# Autodesk Inventor assembly: Tamale Assembly Plate 0p625in with PCB
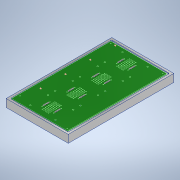
[picture p0: Inventor's stored thumbnail of the model, 180x180]
Saved by Autodesk Inventor 2022 (Build 260153000, 153)
## iProperties
Created: 2022-01-14
Part Number: Tamale Assembly Plate 0p625in with PCB
Document SubType Name: Assembly
Designer: Caleb
Author: Caleb
## Documents named in this file (3)
- C:\Users\Caleb\Desktop\nebraska-silicon-lab\Hardware\ETL\Module Assembly\Tamale Assembly Plate V2\Tamale Assembly Plate 0p625in with PCB.iam
- C:\Users\Caleb\Desktop\nebraska-silicon-lab\Hardware\ETL\Module Assembly\Tamale Assembly Plate V2\Tamale Assembly Plate 0p625in.ipt
- C:\Users\Caleb\Desktop\nebraska-silicon-lab\Hardware\ETL\Module Assembly\Tamale Assembly Plate V2\etl_assembly_plate_pcb_v1.1\etl_assembly_plate_pcb_v1.iam
## Components (2 placed, 2 different names)
1. Tamale Assembly Plate 0p625in:1 — Mate:1, Angle:1, Insert:1
2. etl_assembly_plate_pcb_v1:1 [sub-assembly] — Mate:1, Angle:1, Insert:1
## Relationships (3: Mate 1, Angle 1, Insert 1)
- Mate:1: Tamale Assembly Plate 0p625in:1 ↔ etl_assembly_plate_pcb_v1:1
- Angle:1 (0 deg): Tamale Assembly Plate 0p625in:1 ↔ etl_assembly_plate_pcb_v1:1
- Insert:1: Tamale Assembly Plate 0p625in:1 ↔ etl_assembly_plate_pcb_v1:1
